# Autodesk Inventor assembly: 足回り試作2020v2
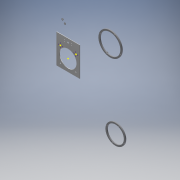
[picture p0: Inventor's stored thumbnail of the model, 180x180]
Saved by Autodesk Inventor 2019 (Build 230136000, 136)
## iProperties
Created: 2020-10-19
Part Number: 足回り試作2020v2
Material: 一般
Document SubType Name: Assembly
Designer: zhept
Author: zhept
## Documents named in this file (5)
- C:\Users\zhept\OneDrive\大学\rrst\足回り2020\足回り試作2020v2.iam
- C:\Users\zhept\OneDrive\大学\rrst\足回り2020\足回り試作2020_v1\ベアリング板.ipt
- C:\Users\zhept\OneDrive\大学\rrst\足回り2020\ワッシャー_M8＿3.2mm.ipt
- C:\Users\zhept\OneDrive\大学\rrst\足回り2020\足回り試作2020_v1\ベアリング 外側.ipt
- C:\Users\zhept\OneDrive\大学\rrst\足回り2020\足回り試作2020_v1\ベアリング 内側.ipt
## Components (7 placed, 4 different names)
1. ベアリング板:1 — メイト:1, 角度:1
2. ワッシャー_M8＿3.2mm:1
3. ワッシャー_M8＿3.2mm:2
4. ワッシャー_M8＿3.2mm:3 — 挿入:1
5. ワッシャー_M8＿3.2mm:4
6. ベアリング 外側:1 — 挿入:1
7. ベアリング 内側:1
## Relationships (4: Mate 1, Angle 1, Flush 1, Insert 1)
- メイト:1 [Mate]: ベアリング板:1
- 角度:1 [Angle] (0 deg): ベアリング板:1
- [Flush]: ベアリング 外側:1 ↔ ベアリング 内側:1
- 挿入:1 [Insert]: ワッシャー_M8＿3.2mm:3 ↔ ベアリング 外側:1
## Named parameters: d7_d6 = 0 mm
